# Autodesk Inventor assembly: KneeSlashCutCrankUnit
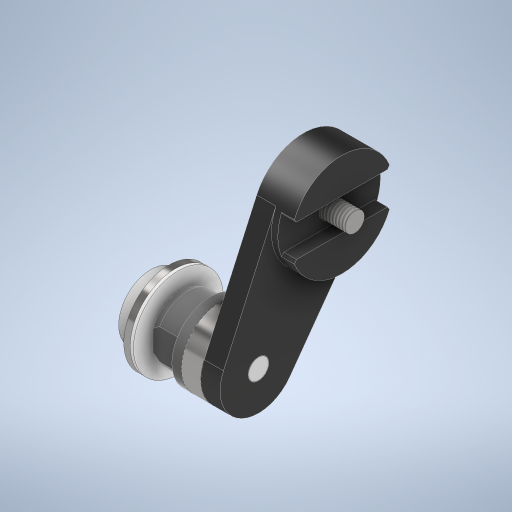
[picture p0: Inventor's stored thumbnail of the model, 512x512]
Saved by Autodesk Inventor 2024.2 (Build 282272000, 272)
## iProperties
Created: 2024-01-06
Part Number: KneeSlashCutCrankUnit
Document SubType Name: Assembly
Designer: Masato Kubotera
Author: Masato Kubotera
## Documents named in this file (8)
- C:\Users\masato\OneDrive - Chiba Institute of Technology\CIT Brains\RoboCup2024\Mechanic\SUSTAINA-OP2\NativeFiles\Boby\LowerLimb\Legs\Knees\KneeSlashCutCrankUnit.iam
- C:\Users\masato\OneDrive - Chiba Institute of Technology\CIT Brains\RoboCup2024\Mechanic\SUSTAINA-OP2\NativeFiles\Boby\COTS\Washers\Metal\UUW-0412-30H.ipt
- C:\Users\masato\OneDrive - Chiba Institute of Technology\CIT Brains\RoboCup2024\Mechanic\SUSTAINA-OP2\NativeFiles\Boby\COTS\Bushes\LED-0606.ipt
- C:\Users\masato\OneDrive - Chiba Institute of Technology\CIT Brains\RoboCup2024\Mechanic\SUSTAINA-OP2\NativeFiles\Boby\COTS\Screws\ScrewsWithShoulder\DBSY4-8-6.ipt
- C:\Users\masato\OneDrive - Chiba Institute of Technology\CIT Brains\RoboCup2024\Mechanic\SUSTAINA-OP2\NativeFiles\Boby\CommonDesignedComponents\SlashCutLongCrankFrame.ipt
- C:\Users\masato\OneDrive - Chiba Institute of Technology\CIT Brains\RoboCup2024\Mechanic\SUSTAINA-OP2\NativeFiles\Boby\COTS\Washers\Metal\UUW-0614-10H.ipt
- C:\Users\masato\OneDrive - Chiba Institute of Technology\CIT Brains\RoboCup2024\Mechanic\SUSTAINA-OP2\NativeFiles\Boby\COTS\Washers\Resin\TT-0614-05.ipt
- C:\Users\masato\OneDrive - Chiba Institute of Technology\CIT Brains\RoboCup2024\Mechanic\SUSTAINA-OP2\NativeFiles\Boby\COTS\Screws\CapScrew\UC-0308.ipt
## Components (7 placed, 7 different names)
1. SlashCutLongCrankFrame:1 — Mate:1, Angle:3, Flush:1, Insert:1, Insert:3
2. UUW-0614-10H:1 — Insert:4, Insert:5
3. TT-0614-05:1 — Insert:4
4. UUW-0412-30H:1 — Insert:1, Insert:2, Insert:6
5. LED-0606:1 — Insert:2, Angle:1
6. UC-0308:1 — Insert:3
7. DBSY4-8-6:1 — Insert:5, Insert:6
## Relationships (10: Insert 6, Angle 2, Mate 1, Flush 1)
- Mate:1: SlashCutLongCrankFrame:1
- Angle:3 (0 deg): SlashCutLongCrankFrame:1
- Flush:1 (20.25 mm): SlashCutLongCrankFrame:1
- Insert:1: SlashCutLongCrankFrame:1 ↔ UUW-0412-30H:1
- Insert:2: UUW-0412-30H:1 ↔ LED-0606:1
- Angle:1 (0 deg): LED-0606:1
- Insert:3: SlashCutLongCrankFrame:1 ↔ UC-0308:1
- Insert:4: UUW-0614-10H:1 ↔ TT-0614-05:1
- Insert:5: UUW-0614-10H:1 ↔ DBSY4-8-6:1
- Insert:6: UUW-0412-30H:1 ↔ DBSY4-8-6:1
